# Autodesk Inventor assembly: Assembly
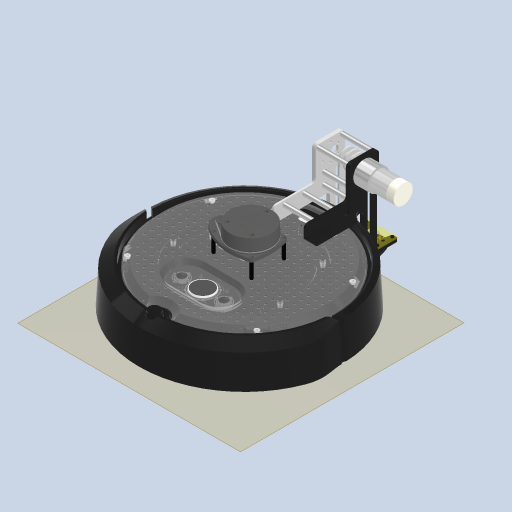
[picture p0: Inventor's stored thumbnail of the model, 512x512]
Saved by Autodesk Inventor 2024 (Build 280153000, 153)
## iProperties
Created: 2023-11-21
Part Number: Assembly
Document SubType Name: Assembly
Designer: Greg
Author: Greg
## Documents named in this file (4)
- C:\Users\Greg\Documents\Inventor\Capstone\Assembly.iam
- C:\Users\Greg\Documents\Inventor\Capstone\iRobot_Create_3_Public_Model\iRobot_Create_3_Public_Model.iam
- C:\Users\Greg\Documents\Inventor\Capstone\RPLIDAR A1M8\RPLIDAR A1M8.iam
- C:\Users\Greg\Documents\Inventor\Capstone\Chalk Applicator\Chalk Applicator.iam
## Components (3 placed, 3 different names)
1. iRobot_Create_3_Public_Model:1 [sub-assembly] — Angle:1, Tangent:1, Insert:1, Mate:1, Mate:2, Mate:3
2. RPLIDAR A1M8:1 [sub-assembly] — Insert:1
3. Chalk Applicator:1 [sub-assembly] — Mate:1, Mate:2, Mate:3
## Relationships (6: Mate 3, Angle 1, Tangent 1, Insert 1)
- Angle:1 (0 deg): iRobot_Create_3_Public_Model:1
- Tangent:1: iRobot_Create_3_Public_Model:1
- Insert:1: iRobot_Create_3_Public_Model:1 ↔ RPLIDAR A1M8:1
- Mate:1: iRobot_Create_3_Public_Model:1 ↔ Chalk Applicator:1
- Mate:2: iRobot_Create_3_Public_Model:1 ↔ Chalk Applicator:1
- Mate:3: iRobot_Create_3_Public_Model:1 ↔ Chalk Applicator:1
